# Autodesk Inventor assembly: ontel_installed
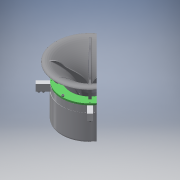
[picture p0: Inventor's stored thumbnail of the model, 180x180]
Saved by Autodesk Inventor 2016 SP1 (Build 200210100, 210)
## iProperties
Created: 2015-12-11
Part Number: ontel_installed
Document SubType Name: Assembly
Designer: ddeboer
Author: ddeboer
## Documents named in this file (5)
- C:\Users\ddeboer\Desktop\leuschner-cad\ontel_installed.iam
- C:\Users\ddeboer\Desktop\leuschner-cad\onTelMountingAssy.iam
- C:\Users\ddeboer\Desktop\leuschner-cad\Quad Assy.iam
- C:\Users\ddeboer\Desktop\leuschner-cad\qtr20_75.ipt
- C:\Users\ddeboer\Desktop\leuschner-cad\cover.ipt
## Components (7 placed, 4 different names)
1. onTelMountingAssy:1 [sub-assembly] — Insert:1, Insert:2, Insert:7
2. Quad Assy:1 [sub-assembly] — Insert:1, Insert:2, Insert:3, Insert:4, Insert:5, Insert:6
3. qtr20_75:1 — Insert:3
4. qtr20_75:2 — Insert:6
5. qtr20_75:3 — Insert:4
6. qtr20_75:4 — Insert:5
7. cover:1 — Insert:7
## Relationships (7: Insert 7)
- Insert:1: onTelMountingAssy:1 ↔ Quad Assy:1
- Insert:2: onTelMountingAssy:1 ↔ Quad Assy:1
- Insert:3: Quad Assy:1 ↔ qtr20_75:1
- Insert:4: Quad Assy:1 ↔ qtr20_75:3
- Insert:5: Quad Assy:1 ↔ qtr20_75:4
- Insert:6: Quad Assy:1 ↔ qtr20_75:2
- Insert:7 (-12.7 mm): onTelMountingAssy:1 ↔ cover:1
